# Autodesk Inventor assembly: Subsystem_1_Hopper
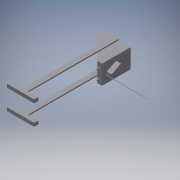
[picture p0: Inventor's stored thumbnail of the model, 180x180]
Saved by Autodesk Inventor 2019.4 (Build 234330000, 330)
## iProperties
Created: 2020-02-13
Part Number: Subsystem_1_Hopper
Document SubType Name: Assembly
Designer: ASUS
Author: ASUS
## Documents named in this file (4)
- C:\Users\Admin\Desktop\Exploration\Subsystem_1_Hopper.iam
- C:\Users\Admin\Desktop\Exploration\hopper 2.ipt
- C:\Users\Admin\Desktop\Exploration\Part2.ipt
- C:\Users\Admin\Desktop\Exploration\hopper stand.ipt
## Components (5 placed, 3 different names)
1. hopper 2:1 — Rigid:1, Rigid:2, Rigid:4
2. hopper 2:2 — Rigid:1, Rigid:3
3. Part2:1 — Rigid:2
4. hopper stand:1 — Rigid:4
5. hopper stand:2 — Rigid:3
## Relationships (4: WeldJoint 4)
- Rigid:1 [WeldJoint]: hopper 2:1 ↔ hopper 2:2
- Rigid:2 [WeldJoint]: hopper 2:1 ↔ Part2:1
- Rigid:3 [WeldJoint]: hopper 2:2 ↔ hopper stand:2
- Rigid:4 [WeldJoint]: hopper 2:1 ↔ hopper stand:1
